# Autodesk Inventor assembly: window_and_tee
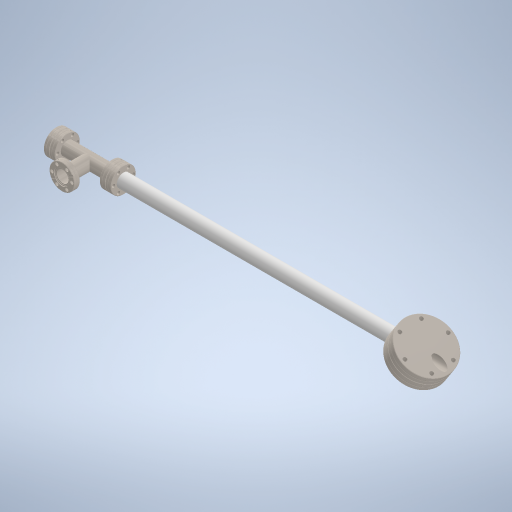
[picture p0: Inventor's stored thumbnail of the model, 512x512]
Saved by Autodesk Inventor 2024 (Build 280153000, 153)
## iProperties
Created: 2024-11-08
Part Number: window_and_tee
Document SubType Name: Assembly
Designer: Andreas Weber
Author: Andreas Weber
## Documents named in this file (4)
- C:\Users\Andreas Weber\Desktop\Upload for Github\window_and_tee.iam
- C:\Users\Andreas Weber\Desktop\Upload for Github\tee_CF16.ipt
- C:\Users\Andreas Weber\Desktop\Upload for Github\Flange_tube.iam
- C:\Users\Andreas Weber\Desktop\Upload for Github\weld_flange_CF16.ipt
## Components (4 placed, 3 different names)
1. Flange_tube:1 [sub-assembly] — Einfügen:1
2. tee_CF16:1 — Drehbar:1, Einfügen:1, Drehbar:3
3. weld_flange_CF16:1 — Drehbar:1
4. weld_flange_CF16:3 — Drehbar:3
## Relationships (3: RevoluteJoint 2, Insert 1)
- Drehbar:1 [RevoluteJoint]: tee_CF16:1 ↔ weld_flange_CF16:1
- Einfügen:1 [Insert]: Flange_tube:1 ↔ tee_CF16:1
- Drehbar:3 [RevoluteJoint]: tee_CF16:1 ↔ weld_flange_CF16:3
